# Autodesk Inventor assembly: stackBothSides
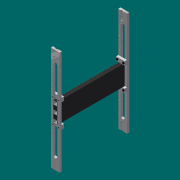
[picture p0: Inventor's stored thumbnail of the model, 180x180]
Saved by Autodesk Inventor 2016 SP1 (Build 200210100, 210)
## iProperties
Created: 2016-02-15
Part Number: stackBothSides
Document SubType Name: Assembly
Designer: sawai
Author: sawai
## Documents named in this file (8)
- C:\Users\Sawaiz\OneDrive\projects\modularHodoscope\fingerMount\stackBothSides.iam
- C:\Users\Sawaiz\OneDrive\projects\modularHodoscope\dependency\scintillatorPanel\scintillatorPanel.iam
- C:\Users\Sawaiz\OneDrive\projects\modularHodoscope\fingerMount\coluredSpacer.ipt
- C:\Users\Sawaiz\OneDrive\projects\modularHodoscope\fingerMount\mppcMount.ipt
- C:\Users\Sawaiz\OneDrive\projects\modularHodoscope\fingerMount\suppourtBlock.ipt
- C:\Users\Sawaiz\OneDrive\projects\modularHodoscope\hardware\4-40x0.5in.ipt
- C:\Users\Sawaiz\OneDrive\projects\modularHodoscope\modularHodoscope.xlsx
- C:\Users\Sawaiz\OneDrive\projects\modularHodoscope\dependency\scintillatorPanel\scintillator.xlsx
## Components (22 placed, 5 different names)
1. mppcMount:1 — Mate:7, Flush:21, Flush:22, Symmetry:1, Symmetry:2, Symmetry:3, Mate:9, Flush:25, Mate:10, Flush:28, Angle:1, Mate:28, Flush:37, Flush:38, Flush:39, Flush:41
2. mppcMount:2 — Flush:21, Flush:22, Symmetry:1, Symmetry:2, Symmetry:3, Mate:8, Flush:24, Mate:11, Flush:27, Flush:35
3. suppourtBlock:1 — Mate:11, Flush:27, Flush:29, Mate:18, Mate:19, Mate:25
4. suppourtBlock:2 — Mate:10, Flush:28, Flush:29, Mate:12, Mate:13, Mate:20, Mate:21, Mate:22, Flush:39, Mate:30
5. suppourtBlock:3 — Mate:8, Flush:24, Flush:26, Mate:16, Mate:17, Mate:24
6. suppourtBlock:4 — Mate:9, Flush:25, Flush:26, Mate:14, Mate:15, Mate:23, Mate:30
7. 4-40x0.5in:1 — Flush:32, Mate:19, Mate:25
8. 4-40x0.5in:2 — Flush:32, Mate:18
9. 4-40x0.5in:3 — Mate:12, Flush:34, Mate:21
10. 4-40x0.5in:4 — Mate:13, Flush:34, Mate:20, Mate:22
11. 4-40x0.5in:5 — Mate:16, Flush:31
12. 4-40x0.5in:6 — Mate:17, Flush:31, Mate:24
13. 4-40x0.5in:7 — Mate:15, Flush:33
14. 4-40x0.5in:8 — Mate:14, Flush:33, Mate:23
15. coluredSpacer:1 — Mate:7, Flush:36, Mate:29
16. coluredSpacer:2
17. coluredSpacer:3
18. scintillatorPanel:1 [sub-assembly] — Angle:1, Flush:35, Mate:28, Flush:36, Mate:29, Flush:37, Flush:38, Flush:40, Mate:31
19. scintillatorPanel:4 [sub-assembly]
20. scintillatorPanel:6 [sub-assembly]
21. scintillatorPanel:3 [sub-assembly] — Flush:40, Flush:41, Mate:31
22. scintillatorPanel:5 [sub-assembly]
## Component patterns: (3 elements, first: coluredSpacer:1), (3 elements, first: scintillatorPanel:1), (2 elements, first: scintillatorPanel:3)
## Relationships (46: Mate 23, Flush 19, Symmetry 3, Angle 1)
- Mate:7: mppcMount:1 ↔ coluredSpacer:1
- Flush:21: mppcMount:1 ↔ mppcMount:2
- Flush:22: mppcMount:1 ↔ mppcMount:2
- Symmetry:1: mppcMount:1 ↔ mppcMount:2
- Symmetry:2: mppcMount:1 ↔ mppcMount:2
- Symmetry:3: mppcMount:1 ↔ mppcMount:2
- Mate:8: mppcMount:2 ↔ suppourtBlock:3
- Flush:24: mppcMount:2 ↔ suppourtBlock:3
- Mate:9: mppcMount:1 ↔ suppourtBlock:4
- Flush:25: mppcMount:1 ↔ suppourtBlock:4
- Flush:26: suppourtBlock:3 ↔ suppourtBlock:4
- Mate:10: mppcMount:1 ↔ suppourtBlock:2
- Mate:11: mppcMount:2 ↔ suppourtBlock:1
- Flush:27: mppcMount:2 ↔ suppourtBlock:1
- Flush:28: mppcMount:1 ↔ suppourtBlock:2
- Flush:29: suppourtBlock:1 ↔ suppourtBlock:2
- Mate:12: suppourtBlock:2 ↔ 4-40x0.5in:3
- Mate:13: suppourtBlock:2 ↔ 4-40x0.5in:4
- Mate:14: suppourtBlock:4 ↔ 4-40x0.5in:8
- Mate:15: suppourtBlock:4 ↔ 4-40x0.5in:7
- Mate:16: suppourtBlock:3 ↔ 4-40x0.5in:5
- Mate:17: suppourtBlock:3 ↔ 4-40x0.5in:6
- Flush:31: 4-40x0.5in:5 ↔ 4-40x0.5in:6
- Flush:32: 4-40x0.5in:1 ↔ 4-40x0.5in:2
- Flush:33: 4-40x0.5in:7 ↔ 4-40x0.5in:8
- Flush:34: 4-40x0.5in:3 ↔ 4-40x0.5in:4
- Mate:18: suppourtBlock:1 ↔ 4-40x0.5in:2
- Mate:19: suppourtBlock:1 ↔ 4-40x0.5in:1
- Mate:20: suppourtBlock:2 ↔ 4-40x0.5in:4
- Mate:21: suppourtBlock:2 ↔ 4-40x0.5in:3
- Mate:22: suppourtBlock:2 ↔ 4-40x0.5in:4
- Mate:23: suppourtBlock:4 ↔ 4-40x0.5in:8
- Mate:24: suppourtBlock:3 ↔ 4-40x0.5in:6
- Mate:25: suppourtBlock:1 ↔ 4-40x0.5in:1
- Angle:1 (0 deg): mppcMount:1 ↔ scintillatorPanel:1
- Flush:35: mppcMount:2 ↔ scintillatorPanel:1
- Mate:28: mppcMount:1 ↔ scintillatorPanel:1
- Flush:36: coluredSpacer:1 ↔ scintillatorPanel:1
- Mate:29: coluredSpacer:1 ↔ scintillatorPanel:1
- Flush:37: mppcMount:1 ↔ scintillatorPanel:1
- Flush:38 (150 mm): mppcMount:1 ↔ scintillatorPanel:1
- Flush:39 (115.752 mm): mppcMount:1 ↔ suppourtBlock:2
- Mate:30 (57.08 mm): suppourtBlock:2 ↔ suppourtBlock:4
- Flush:40: scintillatorPanel:1 ↔ scintillatorPanel:3
- Flush:41: mppcMount:1 ↔ scintillatorPanel:3
- Mate:31: scintillatorPanel:1 ↔ scintillatorPanel:3
## Named parameters: fingerCount = 5, mppcMountThickness = 6.35 mm, opticalFiberDiameter = 1 mm, scintillatorThickness = 10 mm, opticalFiberClearence = 0.071 mm, scintillatorEdgeClearence = 3 mm, scintillatorWidth = 10 mm, scintillatorHeight = 200 mm, shallowTrackDepth = 1.142 mm, deepTrackDepth = 5.571 mm, fiberEdgeOffsett = 5 mm, curvatureRadius = 90 mm, silveringThickness = 0.2 mm, rubberizedCoating = 0.0508, depth = 100 mm, height = 300 mm, width = 300 mm, facingThickness = 12.7 mm, facingGasketThickness = 1.5875 mm, mppcMountDepth = 6.35 mm, ShallowTrackDepth = 1.142 mm, LoopSmallTrackDiameter = 90 mm, LoopLargeTrackRatio = 1.1, ScintillatorHeight = 200 mm, MountingScrewOffsett = 9 mm, LoopLength = 140 mm, FiberEdgeOffsett = 5 mm, DeepTrackDepth = 5.571 mm, FiberSensorClerence = 0.5 mm, ScintillatorEdgeClearence = 3 mm, OpticalFiberClearence = 0.071 mm, ScintillatorThickness = 10 mm, ScintillatorWidth = 10 mm
note: some values were not read from the file. Shown as the stored number, unit unknown: "rubberizedCoating".
